# Autodesk Inventor assembly: IntakeAssembly-ver1-1111-2020
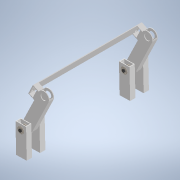
[picture p0: Inventor's stored thumbnail of the model, 180x180]
Saved by Autodesk Inventor 2021 (Build 250183000, 183)
## iProperties
Created: 2020-01-11
Part Number: IntakeAssembly-ver1-1111-2020
Document SubType Name: Assembly
Designer: Power Hawks CADD
Author: Power Hawks CADD
## Documents named in this file (8)
- C:\Users\con_c_000\Documents\GitHub\RoboticsCad1111\PHRC CADD\2020 Infinite Recharge\Final Robot Assembly\IntakeAssembly-ver1-1111-2020.iam
- C:\Users\con_c_000\Documents\GitHub\RoboticsCad1111\PHRC CADD\2020 Infinite Recharge\Intake\Parts\WristBarr.ver1-1111-2020.ipt
- C:\Users\con_c_000\Documents\GitHub\RoboticsCad1111\PHRC CADD\Resources\VEXpro Resources\Bearings\0.5inHexFlangedBearing(1.125inx0.313in)-1111-2016.ipt
- C:\Users\con_c_000\Documents\GitHub\RoboticsCad1111\PHRC CADD\2020 Infinite Recharge\Intake\Parts\1x2AluminumSpacer.ver1-1111-2020.ipt
- C:\Users\con_c_000\Documents\GitHub\RoboticsCad1111\PHRC CADD\2020 Infinite Recharge\Intake\Parts\OverheadSupportBar.ver1-1111-2020.ipt
- C:\Users\con_c_000\Documents\GitHub\RoboticsCad1111\PHRC CADD\2020 Infinite Recharge\Intake\Parts\WristFulcrum.ver-1111-2020.ipt
- C:\Users\con_c_000\Documents\GitHub\RoboticsCad1111\PHRC CADD\2020 Infinite Recharge\Intake\Parts\0.5inThunderHexShaft4in-1111-2020.ipt
- C:\Users\con_c_000\Documents\GitHub\RoboticsCad1111\PHRC CADD\Resources\VEXpro Resources\Spacers\0.125inAcetalSpacer(0.5inHex)-1111-2016.ipt
## Components (27 placed, 7 different names)
1. WristBarr.ver1-1111-2020:1 — Flush:2, Mate:25, Flush:3, Mate:26, Cylindrical:26, Mate:29, Rigid:1
2. WristBarr.ver1-1111-2020:2 — Flush:2, Mate:28, Flush:6, Rigid:2, Rigid:3
3. OverheadSupportBar.ver1-1111-2020:1 — Mate:27, Flush:4, Flush:5, Flush:7
4. 1x2AluminumSpacer.ver1-1111-2020:1 — Mate:25, Flush:3, Mate:26, Mate:27, Flush:4, Flush:5
5. 1x2AluminumSpacer.ver1-1111-2020:2 — Mate:28, Flush:6, Flush:7
6. 0.5inHexFlangedBearing(1.125inx0.313in)-1111-2016:9 — Rigid:2, Mate:36
7. 0.5inHexFlangedBearing(1.125inx0.313in)-1111-2016:10 — Cylindrical:26, Mate:29, Cylindrical:28, Mate:32
8. 0.5inHexFlangedBearing(1.125inx0.313in)-1111-2016:11 — Rigid:3, Cylindrical:27, Mate:37
9. 0.5inHexFlangedBearing(1.125inx0.313in)-1111-2016:12 — Rigid:1, Mate:34
10. WristFulcrum.ver-1111-2020:1 — Rotational:1, Rotational:2, Flush:9, Flush:10
11. WristFulcrum.ver-1111-2020:2 — Rotational:3, Rotational:4, Flush:9
12. WristFulcrum.ver-1111-2020:3 — Rotational:5, Rotational:6, Flush:10, Flush:11
13. WristFulcrum.ver-1111-2020:4 — Rotational:7, Rotational:8, Flush:11
14. 0.5inHexFlangedBearing(1.125inx0.313in)-1111-2016:13 — Rotational:1, Cylindrical:30, Mate:35
15. 0.5inHexFlangedBearing(1.125inx0.313in)-1111-2016:14 — Rotational:4, Cylindrical:29, Mate:33
16. 0.5inHexFlangedBearing(1.125inx0.313in)-1111-2016:15 — Rotational:2
17. 0.5inHexFlangedBearing(1.125inx0.313in)-1111-2016:16 — Rotational:3, Flush:12
18. 0.5inHexFlangedBearing(1.125inx0.313in)-1111-2016:17 — Rotational:6, Flush:13
19. 0.5inHexFlangedBearing(1.125inx0.313in)-1111-2016:18 — Rotational:8
20. 0.5inHexFlangedBearing(1.125inx0.313in)-1111-2016:19 — Rotational:5, Cylindrical:32, Mate:38
21. 0.5inHexFlangedBearing(1.125inx0.313in)-1111-2016:20 — Rotational:7, Cylindrical:31, Mate:39
22. 0.5inThunderHexShaft4in-1111-2020:1 — Cylindrical:28, Cylindrical:29, Cylindrical:30, Cylindrical:33, Cylindrical:34, Flush:12
23. 0.5inThunderHexShaft4in-1111-2020:2 — Cylindrical:27, Cylindrical:31, Cylindrical:32, Cylindrical:35, Cylindrical:36, Flush:13
24. 0.125inAcetalSpacer(0.5inHex)-1111-2016:1 — Cylindrical:33, Mate:32, Mate:33
25. 0.125inAcetalSpacer(0.5inHex)-1111-2016:2 — Cylindrical:34, Mate:34, Mate:35
26. 0.125inAcetalSpacer(0.5inHex)-1111-2016:3 — Cylindrical:36, Mate:36, Mate:38
27. 0.125inAcetalSpacer(0.5inHex)-1111-2016:4 — Cylindrical:35, Mate:37, Mate:39
## Relationships (46: Mate 13, Flush 11, CylindricalJoint 11, RevoluteJoint 8, WeldJoint 3)
- Flush:2: WristBarr.ver1-1111-2020:1 ↔ WristBarr.ver1-1111-2020:2
- Mate:25: WristBarr.ver1-1111-2020:1 ↔ 1x2AluminumSpacer.ver1-1111-2020:1
- Flush:3: WristBarr.ver1-1111-2020:1 ↔ 1x2AluminumSpacer.ver1-1111-2020:1
- Mate:26: WristBarr.ver1-1111-2020:1 ↔ 1x2AluminumSpacer.ver1-1111-2020:1
- Mate:27: OverheadSupportBar.ver1-1111-2020:1 ↔ 1x2AluminumSpacer.ver1-1111-2020:1
- Flush:4: OverheadSupportBar.ver1-1111-2020:1 ↔ 1x2AluminumSpacer.ver1-1111-2020:1
- Flush:5: OverheadSupportBar.ver1-1111-2020:1 ↔ 1x2AluminumSpacer.ver1-1111-2020:1
- Mate:28: WristBarr.ver1-1111-2020:2 ↔ 1x2AluminumSpacer.ver1-1111-2020:2
- Flush:6: WristBarr.ver1-1111-2020:2 ↔ 1x2AluminumSpacer.ver1-1111-2020:2
- Flush:7: OverheadSupportBar.ver1-1111-2020:1 ↔ 1x2AluminumSpacer.ver1-1111-2020:2
- Cylindrical:26: WristBarr.ver1-1111-2020:1 ↔ 0.5inHexFlangedBearing(1.125inx0.313in)-1111-2016:10
- Mate:29: WristBarr.ver1-1111-2020:1 ↔ 0.5inHexFlangedBearing(1.125inx0.313in)-1111-2016:10
- Rigid:1 [WeldJoint]: WristBarr.ver1-1111-2020:1 ↔ 0.5inHexFlangedBearing(1.125inx0.313in)-1111-2016:12
- Rigid:2 [WeldJoint]: WristBarr.ver1-1111-2020:2 ↔ 0.5inHexFlangedBearing(1.125inx0.313in)-1111-2016:9
- Rigid:3 [WeldJoint]: WristBarr.ver1-1111-2020:2 ↔ 0.5inHexFlangedBearing(1.125inx0.313in)-1111-2016:11
- Rotational:1 [RevoluteJoint]: WristFulcrum.ver-1111-2020:1 ↔ 0.5inHexFlangedBearing(1.125inx0.313in)-1111-2016:13
- Rotational:2 [RevoluteJoint]: WristFulcrum.ver-1111-2020:1 ↔ 0.5inHexFlangedBearing(1.125inx0.313in)-1111-2016:15
- Rotational:3 [RevoluteJoint]: WristFulcrum.ver-1111-2020:2 ↔ 0.5inHexFlangedBearing(1.125inx0.313in)-1111-2016:16
- Rotational:4 [RevoluteJoint]: WristFulcrum.ver-1111-2020:2 ↔ 0.5inHexFlangedBearing(1.125inx0.313in)-1111-2016:14
- Rotational:5 [RevoluteJoint]: WristFulcrum.ver-1111-2020:3 ↔ 0.5inHexFlangedBearing(1.125inx0.313in)-1111-2016:19
- Rotational:6 [RevoluteJoint]: WristFulcrum.ver-1111-2020:3 ↔ 0.5inHexFlangedBearing(1.125inx0.313in)-1111-2016:17
- Rotational:7 [RevoluteJoint]: WristFulcrum.ver-1111-2020:4 ↔ 0.5inHexFlangedBearing(1.125inx0.313in)-1111-2016:20
- Rotational:8 [RevoluteJoint]: WristFulcrum.ver-1111-2020:4 ↔ 0.5inHexFlangedBearing(1.125inx0.313in)-1111-2016:18
- Cylindrical:27: 0.5inHexFlangedBearing(1.125inx0.313in)-1111-2016:11 ↔ 0.5inThunderHexShaft4in-1111-2020:2
- Cylindrical:28: 0.5inHexFlangedBearing(1.125inx0.313in)-1111-2016:10 ↔ 0.5inThunderHexShaft4in-1111-2020:1
- Cylindrical:29: 0.5inHexFlangedBearing(1.125inx0.313in)-1111-2016:14 ↔ 0.5inThunderHexShaft4in-1111-2020:1
- Cylindrical:30: 0.5inHexFlangedBearing(1.125inx0.313in)-1111-2016:13 ↔ 0.5inThunderHexShaft4in-1111-2020:1
- Cylindrical:31: 0.5inHexFlangedBearing(1.125inx0.313in)-1111-2016:20 ↔ 0.5inThunderHexShaft4in-1111-2020:2
- Cylindrical:32: 0.5inHexFlangedBearing(1.125inx0.313in)-1111-2016:19 ↔ 0.5inThunderHexShaft4in-1111-2020:2
- Flush:9: WristFulcrum.ver-1111-2020:1 ↔ WristFulcrum.ver-1111-2020:2
- Flush:10: WristFulcrum.ver-1111-2020:1 ↔ WristFulcrum.ver-1111-2020:3
- Flush:11: WristFulcrum.ver-1111-2020:3 ↔ WristFulcrum.ver-1111-2020:4
- Cylindrical:33: 0.5inThunderHexShaft4in-1111-2020:1 ↔ 0.125inAcetalSpacer(0.5inHex)-1111-2016:1
- Cylindrical:34: 0.5inThunderHexShaft4in-1111-2020:1 ↔ 0.125inAcetalSpacer(0.5inHex)-1111-2016:2
- Mate:32: 0.5inHexFlangedBearing(1.125inx0.313in)-1111-2016:10 ↔ 0.125inAcetalSpacer(0.5inHex)-1111-2016:1
- Mate:33: 0.5inHexFlangedBearing(1.125inx0.313in)-1111-2016:14 ↔ 0.125inAcetalSpacer(0.5inHex)-1111-2016:1
- Mate:34: 0.5inHexFlangedBearing(1.125inx0.313in)-1111-2016:12 ↔ 0.125inAcetalSpacer(0.5inHex)-1111-2016:2
- Mate:35: 0.5inHexFlangedBearing(1.125inx0.313in)-1111-2016:13 ↔ 0.125inAcetalSpacer(0.5inHex)-1111-2016:2
- Flush:12 (4.3815 mm): 0.5inHexFlangedBearing(1.125inx0.313in)-1111-2016:16 ↔ 0.5inThunderHexShaft4in-1111-2020:1
- Cylindrical:35: 0.5inThunderHexShaft4in-1111-2020:2 ↔ 0.125inAcetalSpacer(0.5inHex)-1111-2016:4
- Cylindrical:36: 0.5inThunderHexShaft4in-1111-2020:2 ↔ 0.125inAcetalSpacer(0.5inHex)-1111-2016:3
- Mate:36: 0.5inHexFlangedBearing(1.125inx0.313in)-1111-2016:9 ↔ 0.125inAcetalSpacer(0.5inHex)-1111-2016:3
- Mate:37: 0.5inHexFlangedBearing(1.125inx0.313in)-1111-2016:11 ↔ 0.125inAcetalSpacer(0.5inHex)-1111-2016:4
- Mate:38: 0.5inHexFlangedBearing(1.125inx0.313in)-1111-2016:19 ↔ 0.125inAcetalSpacer(0.5inHex)-1111-2016:3
- Mate:39: 0.5inHexFlangedBearing(1.125inx0.313in)-1111-2016:20 ↔ 0.125inAcetalSpacer(0.5inHex)-1111-2016:4
- Flush:13 (4.3815 mm): 0.5inHexFlangedBearing(1.125inx0.313in)-1111-2016:17 ↔ 0.5inThunderHexShaft4in-1111-2020:2
